# Autodesk Inventor assembly: Turdbot Drivetrain
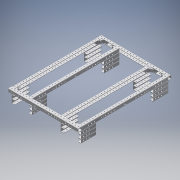
[picture p0: Inventor's stored thumbnail of the model, 180x180]
Saved by Autodesk Inventor 2016 (Build 200138000, 138)
## iProperties
Created: 2016-01-13
Part Number: Turdbot Drivetrain
Document SubType Name: Assembly
Designer: Administrator
Author: Administrator
## Documents named in this file (4)
- C:\Users\Administrator\Desktop\3192CAD\InitialRobotProto\Turdbot Drivetrain.iam
- C:\Users\Administrator\Desktop\3192CAD\InitialRobotProto\DBK_C-Channel_am-2222.ipt
- C:\Users\Administrator\Desktop\3192CAD\InitialRobotProto\DBK_CornerConnect_am-0212.ipt
- C:\Users\Administrator\Desktop\3192CAD\InitialRobotProto\WheelMountStack.iam
## Components (20 placed, 3 different names)
1. DBK_C-Channel_am-2222:1 — Mate:1, Mate:2, Mate:3, Mate:16, Mate:17, Mate:18, Mate:34, Mate:35, Mate:36, Mate:37, Mate:38, Mate:39
2. DBK_C-Channel_am-2222:2 — Mate:4, Mate:5, Mate:6, Mate:7, Mate:8, Mate:9, Mate:22, Mate:23, Mate:24, Mate:25, Mate:26, Mate:27
3. DBK_C-Channel_am-2222:3 — Mate:19, Mate:20, Mate:21
4. DBK_C-Channel_am-2222:4 — Mate:10, Mate:11, Mate:12, Mate:13, Mate:14, Mate:15, Mate:52, Mate:53, Mate:54, Mate:55, Mate:56, Mate:57
5. DBK_CornerConnect_am-0212:1 — Mate:7, Mate:8, Mate:9, Mate:10, Mate:11, Mate:12
6. DBK_CornerConnect_am-0212:2 — Mate:16, Mate:17, Mate:18
7. DBK_CornerConnect_am-0212:3 — Mate:1, Mate:2, Mate:3, Mate:4, Mate:5, Mate:6
8. DBK_CornerConnect_am-0212:4 — Mate:13, Mate:14, Mate:15, Mate:19, Mate:20, Mate:21
9. DBK_C-Channel_am-2222:5 — Mate:31, Mate:32, Mate:33, Mate:40, Mate:41, Mate:42, Mate:43, Mate:44, Mate:45
10. DBK_C-Channel_am-2222:6 — Mate:28, Mate:29, Mate:30, Mate:46, Mate:47, Mate:48, Mate:49, Mate:50, Mate:51
11. DBK_CornerConnect_am-0212:5 — Mate:22, Mate:23, Mate:24, Mate:31, Mate:32, Mate:33
12. DBK_CornerConnect_am-0212:6 — Mate:25, Mate:26, Mate:27, Mate:28, Mate:29, Mate:30
13. WheelMountStack:1 [sub-assembly] — Mate:40, Mate:41, Mate:42
14. WheelMountStack:2 [sub-assembly] — Mate:46, Mate:47, Mate:48
15. WheelMountStack:3 [sub-assembly] — Mate:34, Mate:35, Mate:36
16. WheelMountStack:4 [sub-assembly] — Mate:37, Mate:38, Mate:39
17. WheelMountStack:5 [sub-assembly] — Mate:43, Mate:44, Mate:45
18. WheelMountStack:6 [sub-assembly] — Mate:49, Mate:50, Mate:51
19. WheelMountStack:7 [sub-assembly] — Mate:52, Mate:53, Mate:54
20. WheelMountStack:8 [sub-assembly] — Mate:55, Mate:56, Mate:57
## Relationships (57: Mate 57)
- Mate:1: DBK_C-Channel_am-2222:1 ↔ DBK_CornerConnect_am-0212:3
- Mate:2: DBK_C-Channel_am-2222:1 ↔ DBK_CornerConnect_am-0212:3
- Mate:3: DBK_C-Channel_am-2222:1 ↔ DBK_CornerConnect_am-0212:3
- Mate:4: DBK_C-Channel_am-2222:2 ↔ DBK_CornerConnect_am-0212:3
- Mate:5: DBK_C-Channel_am-2222:2 ↔ DBK_CornerConnect_am-0212:3
- Mate:6: DBK_C-Channel_am-2222:2 ↔ DBK_CornerConnect_am-0212:3
- Mate:7: DBK_C-Channel_am-2222:2 ↔ DBK_CornerConnect_am-0212:1
- Mate:8: DBK_C-Channel_am-2222:2 ↔ DBK_CornerConnect_am-0212:1
- Mate:9: DBK_C-Channel_am-2222:2 ↔ DBK_CornerConnect_am-0212:1
- Mate:10: DBK_C-Channel_am-2222:4 ↔ DBK_CornerConnect_am-0212:1
- Mate:11: DBK_C-Channel_am-2222:4 ↔ DBK_CornerConnect_am-0212:1
- Mate:12: DBK_C-Channel_am-2222:4 ↔ DBK_CornerConnect_am-0212:1
- Mate:13: DBK_C-Channel_am-2222:4 ↔ DBK_CornerConnect_am-0212:4
- Mate:14: DBK_C-Channel_am-2222:4 ↔ DBK_CornerConnect_am-0212:4
- Mate:15: DBK_C-Channel_am-2222:4 ↔ DBK_CornerConnect_am-0212:4
- Mate:16: DBK_C-Channel_am-2222:1 ↔ DBK_CornerConnect_am-0212:2
- Mate:17: DBK_C-Channel_am-2222:1 ↔ DBK_CornerConnect_am-0212:2
- Mate:18: DBK_C-Channel_am-2222:1 ↔ DBK_CornerConnect_am-0212:2
- Mate:19: DBK_C-Channel_am-2222:3 ↔ DBK_CornerConnect_am-0212:4
- Mate:20: DBK_C-Channel_am-2222:3 ↔ DBK_CornerConnect_am-0212:4
- Mate:21: DBK_C-Channel_am-2222:3 ↔ DBK_CornerConnect_am-0212:4
- Mate:22: DBK_C-Channel_am-2222:2 ↔ DBK_CornerConnect_am-0212:5
- Mate:23: DBK_C-Channel_am-2222:2 ↔ DBK_CornerConnect_am-0212:5
- Mate:24: DBK_C-Channel_am-2222:2 ↔ DBK_CornerConnect_am-0212:5
- Mate:25: DBK_C-Channel_am-2222:2 ↔ DBK_CornerConnect_am-0212:6
- Mate:26: DBK_C-Channel_am-2222:2 ↔ DBK_CornerConnect_am-0212:6
- Mate:27: DBK_C-Channel_am-2222:2 ↔ DBK_CornerConnect_am-0212:6
- Mate:28: DBK_C-Channel_am-2222:6 ↔ DBK_CornerConnect_am-0212:6
- Mate:29: DBK_C-Channel_am-2222:6 ↔ DBK_CornerConnect_am-0212:6
- Mate:30: DBK_C-Channel_am-2222:6 ↔ DBK_CornerConnect_am-0212:6
- Mate:31: DBK_C-Channel_am-2222:5 ↔ DBK_CornerConnect_am-0212:5
- Mate:32: DBK_C-Channel_am-2222:5 ↔ DBK_CornerConnect_am-0212:5
- Mate:33: DBK_C-Channel_am-2222:5 ↔ DBK_CornerConnect_am-0212:5
- Mate:34: DBK_C-Channel_am-2222:1 ↔ WheelMountStack:3
- Mate:35: DBK_C-Channel_am-2222:1 ↔ WheelMountStack:3
- Mate:36: DBK_C-Channel_am-2222:1 ↔ WheelMountStack:3
- Mate:37: DBK_C-Channel_am-2222:1 ↔ WheelMountStack:4
- Mate:38: DBK_C-Channel_am-2222:1 ↔ WheelMountStack:4
- Mate:39: DBK_C-Channel_am-2222:1 ↔ WheelMountStack:4
- Mate:40: DBK_C-Channel_am-2222:5 ↔ WheelMountStack:1
- Mate:41: DBK_C-Channel_am-2222:5 ↔ WheelMountStack:1
- Mate:42: DBK_C-Channel_am-2222:5 ↔ WheelMountStack:1
- Mate:43: DBK_C-Channel_am-2222:5 ↔ WheelMountStack:5
- Mate:44: DBK_C-Channel_am-2222:5 ↔ WheelMountStack:5
- Mate:45: DBK_C-Channel_am-2222:5 ↔ WheelMountStack:5
- Mate:46: DBK_C-Channel_am-2222:6 ↔ WheelMountStack:2
- Mate:47: DBK_C-Channel_am-2222:6 ↔ WheelMountStack:2
- Mate:48: DBK_C-Channel_am-2222:6 ↔ WheelMountStack:2
- Mate:49: DBK_C-Channel_am-2222:6 ↔ WheelMountStack:6
- Mate:50: DBK_C-Channel_am-2222:6 ↔ WheelMountStack:6
- Mate:51: DBK_C-Channel_am-2222:6 ↔ WheelMountStack:6
- Mate:52: DBK_C-Channel_am-2222:4 ↔ WheelMountStack:7
- Mate:53: DBK_C-Channel_am-2222:4 ↔ WheelMountStack:7
- Mate:54: DBK_C-Channel_am-2222:4 ↔ WheelMountStack:7
- Mate:55: DBK_C-Channel_am-2222:4 ↔ WheelMountStack:8
- Mate:56: DBK_C-Channel_am-2222:4 ↔ WheelMountStack:8
- Mate:57: DBK_C-Channel_am-2222:4 ↔ WheelMountStack:8
